# Autodesk Inventor assembly: 付け根_1
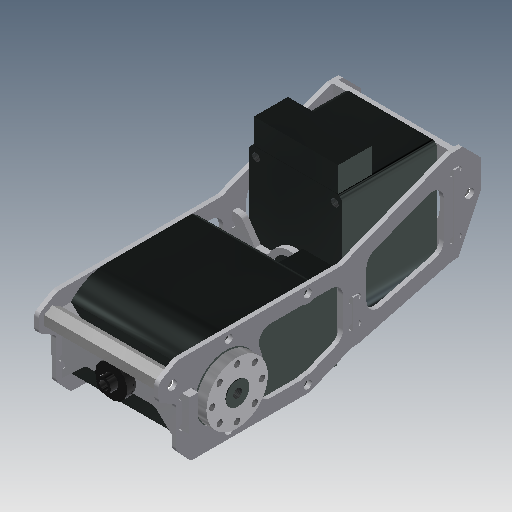
[picture p0: Inventor's stored thumbnail of the model, 512x512]
Saved by Autodesk Inventor 2017.3 (Build 213256000, 256)
## iProperties
Created: 2016-04-27
Part Number: 付け根_1
Document SubType Name: Assembly
Designer: hiroaki
Mass: 227.878 g
Surface Area: 377.938 cm^2
Volume: 115.318 cm^3
Density: 1.97609 g/cm^3
Author: hiroaki
## Documents named in this file (12)
- C:\Users\haya\Desktop\GankenKun0_5\下半身\足首\足首_1_MIR.iam
- C:\Users\haya\Desktop\GankenKun0_5\既製品\B3M11xx.ipt
- C:\Users\haya\Desktop\GankenKun0_5\既製品\free_horn.ipt
- C:\Users\haya\Desktop\GankenKun0_5\下半身\足首\足首_メインフレーム_1_1.ipt
- C:\Users\haya\Desktop\GankenKun0_5\下半身\足首\足首_サブフレーム_1_1.ipt
- C:\Users\haya\Desktop\GankenKun0_5\下半身\足首\足首_サブフレーム_1_2.ipt
- C:\Users\haya\Desktop\GankenKun0_5\下半身\足首\足首_メインフレーム_1_1_MIR.ipt
- C:\Users\haya\Desktop\GankenKun0_5\下半身\足首\足首_サブフレーム_1_3.ipt
- C:\Users\haya\Desktop\GankenKun0_5\下半身\足裏\足裏_サブフレーム_1_2.ipt
- C:\Users\haya\Desktop\GankenKun0_5\既製品\B3M10xx.ipt
- C:\Users\haya\Desktop\GankenKun0_5\既製品\ASU-340.ipt
- C:\Users\haya\Desktop\GankenKun0_5\既製品\CC-0311-08B.ipt
## Components (12 placed, 10 different names)
1. B3M11xx:1 — 挿入:23, メイト:7, 挿入:41, 挿入:42
2. free_horn:1 — 挿入:23
3. 足首_メインフレーム_1_1:1 — メイト:1, メイト:2, メイト:3, メイト:4, メイト:5, メイト:6, メイト:8, 挿入:42, 挿入:48, 挿入:49
4. 足首_サブフレーム_1_1:1 — メイト:1, メイト:2, メイト:3, 挿入:44, 挿入:45
5. 足首_サブフレーム_1_2:1 — メイト:4, メイト:5, メイト:6, 挿入:46
6. 足首_メインフレーム_1_1_MIR:1 — メイト:9, 挿入:41, 挿入:47, 挿入:50, 角度:1, 角度:2
7. 足首_サブフレーム_1_3:1 — メイト:7, メイト:8, メイト:9, 挿入:52
8. 足裏_サブフレーム_1_2:1 — 挿入:51
9. B3M11xx:2 — 挿入:44, 挿入:45, 挿入:46
10. ASU-340:1 — 挿入:47, 挿入:48, 角度:1
11. ASU-340:2 — 挿入:49, 挿入:50, 角度:2
12. CC-0311-08B:1 — 挿入:51, 挿入:52
## Relationships (23: Insert 12, Mate 9, Angle 2)
- 挿入:23 [Insert]: B3M11xx:1 ↔ free_horn:1
- メイト:1 [Mate] (0.025 mm): 足首_メインフレーム_1_1:1 ↔ 足首_サブフレーム_1_1:1
- メイト:2 [Mate]: 足首_メインフレーム_1_1:1 ↔ 足首_サブフレーム_1_1:1
- メイト:3 [Mate] (0.025 mm): 足首_メインフレーム_1_1:1 ↔ 足首_サブフレーム_1_1:1
- メイト:4 [Mate]: 足首_メインフレーム_1_1:1 ↔ 足首_サブフレーム_1_2:1
- メイト:5 [Mate] (0.025 mm): 足首_メインフレーム_1_1:1 ↔ 足首_サブフレーム_1_2:1
- メイト:6 [Mate] (0.025 mm): 足首_メインフレーム_1_1:1 ↔ 足首_サブフレーム_1_2:1
- メイト:7 [Mate]: B3M11xx:1 ↔ 足首_サブフレーム_1_3:1
- メイト:8 [Mate]: 足首_メインフレーム_1_1:1 ↔ 足首_サブフレーム_1_3:1
- メイト:9 [Mate] (0.025 mm): 足首_メインフレーム_1_1_MIR:1 ↔ 足首_サブフレーム_1_3:1
- 挿入:41 [Insert]: B3M11xx:1 ↔ 足首_メインフレーム_1_1_MIR:1
- 挿入:42 [Insert]: B3M11xx:1 ↔ 足首_メインフレーム_1_1:1
- 挿入:44 [Insert]: 足首_サブフレーム_1_1:1 ↔ B3M11xx:2
- 挿入:45 [Insert]: 足首_サブフレーム_1_1:1 ↔ B3M11xx:2
- 挿入:46 [Insert]: 足首_サブフレーム_1_2:1 ↔ B3M11xx:2
- 挿入:47 [Insert]: 足首_メインフレーム_1_1_MIR:1 ↔ ASU-340:1
- 挿入:48 [Insert]: 足首_メインフレーム_1_1:1 ↔ ASU-340:1
- 挿入:49 [Insert]: 足首_メインフレーム_1_1:1 ↔ ASU-340:2
- 挿入:50 [Insert]: 足首_メインフレーム_1_1_MIR:1 ↔ ASU-340:2
- 角度:1 [Angle] (0 deg): 足首_メインフレーム_1_1_MIR:1 ↔ ASU-340:1
- 角度:2 [Angle] (0 deg): 足首_メインフレーム_1_1_MIR:1 ↔ ASU-340:2
- 挿入:51 [Insert]: 足裏_サブフレーム_1_2:1 ↔ CC-0311-08B:1
- 挿入:52 [Insert]: 足首_サブフレーム_1_3:1 ↔ CC-0311-08B:1
